# Autodesk Inventor assembly: leg
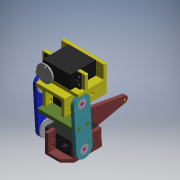
[picture p0: Inventor's stored thumbnail of the model, 180x180]
Saved by Autodesk Inventor 2017 (Build 210142000, 142)
## iProperties
Part Number: leg
Document SubType Name: Assembly
Designer: Alexander Miller
Author: Alexander Miller
## Documents named in this file (9)
- D:\Daten\Documents\Git\Hexapod\3DParts\leg_left.iam
- D:\Daten\Documents\Git\Hexapod\3DParts\Serov_with_arm.iam
- D:\Daten\Documents\Git\Hexapod\3DParts\Upper_leg.ipt
- D:\Daten\Documents\Git\Hexapod\3DParts\ball_bearing.ipt
- D:\Daten\Documents\Git\Hexapod\3DParts\Lower_leg_left.ipt
- D:\Daten\Documents\Git\Hexapod\3DParts\Connector.ipt
- D:\Daten\Documents\Git\Hexapod\3DParts\Middle_leg_a.ipt
- D:\Daten\Documents\Git\Hexapod\3DParts\Middle_leg_b.ipt
- D:\Daten\Documents\Git\Hexapod\3DParts\Middle_leg_c.ipt
## Components (13 placed, 8 different names)
1. Serov_with_arm:1 [sub-assembly] — Rigid:20, Rigid:28
2. Serov_with_arm:2 [sub-assembly] — Rigid:21
3. Upper_leg:1 — Rigid:14, Rigid:20, Rigid:22
4. Upper_leg:2 — Rigid:14, Rigid:21
5. Serov_with_arm:3 [sub-assembly] — Rigid:19, Rigid:29
6. ball_bearing:1 — Rigid:27, Rotational:2
7. ball_bearing:2 — Rigid:26, Rotational:1
8. Lower_leg_left:1 — Rigid:19, Rigid:23
9. Connector:1 — Rigid:23, Rotational:2
10. Connector:2 — Rigid:22, Rotational:1
11. Middle_leg_a:1 — Rigid:28, Rigid:29, Rigid:30
12. Middle_leg_b:1 — Rigid:26, Rigid:27, Rigid:31
13. Middle_leg_c:1 — Rigid:30, Rigid:31
## Relationships (14: WeldJoint 12, RevoluteJoint 2)
- Rigid:14 [WeldJoint]: Upper_leg:1 ↔ Upper_leg:2
- Rigid:19 [WeldJoint]: Serov_with_arm:3 ↔ Lower_leg_left:1
- Rigid:20 [WeldJoint]: Serov_with_arm:1 ↔ Upper_leg:1
- Rigid:21 [WeldJoint]: Serov_with_arm:2 ↔ Upper_leg:2
- Rigid:22 [WeldJoint]: Upper_leg:1 ↔ Connector:2
- Rigid:23 [WeldJoint]: Lower_leg_left:1 ↔ Connector:1
- Rigid:26 [WeldJoint]: ball_bearing:2 ↔ Middle_leg_b:1
- Rigid:27 [WeldJoint]: ball_bearing:1 ↔ Middle_leg_b:1
- Rotational:1 [RevoluteJoint]: ball_bearing:2 ↔ Connector:2
- Rotational:2 [RevoluteJoint]: ball_bearing:1 ↔ Connector:1
- Rigid:28 [WeldJoint]: Serov_with_arm:1 ↔ Middle_leg_a:1
- Rigid:29 [WeldJoint]: Serov_with_arm:3 ↔ Middle_leg_a:1
- Rigid:30 [WeldJoint]: Middle_leg_a:1 ↔ Middle_leg_c:1
- Rigid:31 [WeldJoint]: Middle_leg_b:1 ↔ Middle_leg_c:1
